# Autodesk Inventor assembly: 2-Way Assembly
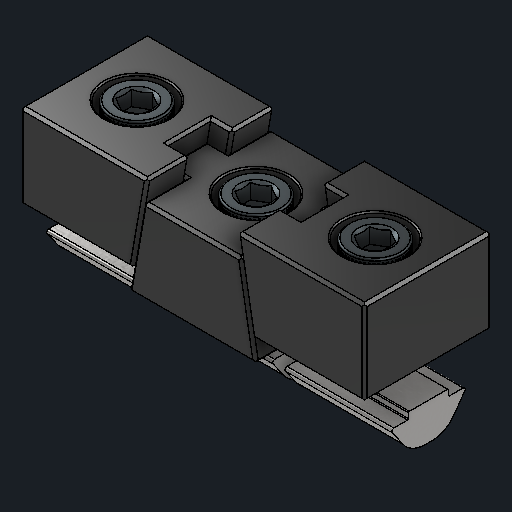
[picture p0: Inventor's stored thumbnail of the model, 512x512]
Saved by Autodesk Inventor 2026.2 (Build 302298000, 298)
## iProperties
Created: 2026-05-18
Part Number: 2-Way Assembly
Document SubType Name: Assembly
Designer: JoshuaEah
Author: JoshuaEah
## Documents named in this file (7)
- C:\Users\JoshuaEah\Documents\GitHub\Designed-Trinkets\Modular Pedalboard\2-Way Assembly.iam
- C:\Users\JoshuaEah\Documents\GitHub\Designed-Trinkets\Modular Pedalboard\2 Way Fixture Base.ipt
- C:\Users\JoshuaEah\Documents\GitHub\Designed-Trinkets\Modular Pedalboard\10-32 T-Nut.ipt
- 10-32 T-Nut.ipt
- C:\Users\JoshuaEah\Documents\GitHub\Designed-Trinkets\Modular Pedalboard\10-32x0.5 SHCS.ipt
- C:\Users\JoshuaEah\Documents\GitHub\Designed-Trinkets\Modular Pedalboard\Fixture Jaw.ipt
- C:\Users\JoshuaEah\Documents\GitHub\Designed-Trinkets\Modular Pedalboard\10-32x0.625 SHCS.ipt
## Components (9 placed, 5 different names)
1. 2 Way Fixture Base:1 — Flush:1, Flush:2
2. 10-32 T-Nut:1
3. 10-32x0.5 SHCS:1
4. 10-32 T-Nut:2
5. 10-32 T-Nut:3
6. Fixture Jaw:1 — Flush:1
7. Fixture Jaw:2 — Flush:2
8. 10-32x0.625 SHCS:1
9. 10-32x0.625 SHCS:2
## Relationships (12: Mate 7, Insert 3, Flush 2)
- [Mate]: 2 Way Fixture Base:1 ↔ 10-32 T-Nut:1
- [Insert]: 2 Way Fixture Base:1 ↔ 10-32x0.5 SHCS:1
- [Mate]: 2 Way Fixture Base:1 ↔ Fixture Jaw:1
- [Mate]: 2 Way Fixture Base:1 ↔ Fixture Jaw:1
- [Mate]: 2 Way Fixture Base:1 ↔ Fixture Jaw:2
- [Mate]: 2 Way Fixture Base:1 ↔ Fixture Jaw:2
- [Mate]: 10-32 T-Nut:3 ↔ Fixture Jaw:1
- [Mate]: 10-32 T-Nut:2 ↔ Fixture Jaw:2
- [Insert]: Fixture Jaw:1 ↔ 10-32x0.625 SHCS:1
- [Insert]: Fixture Jaw:2 ↔ 10-32x0.625 SHCS:2
- Flush:1 (-3.175 mm): 2 Way Fixture Base:1 ↔ Fixture Jaw:1
- Flush:2 (-3.175 mm): 2 Way Fixture Base:1 ↔ Fixture Jaw:2
